# Autodesk Inventor assembly: Carrier Wirebonding Plate Assembly
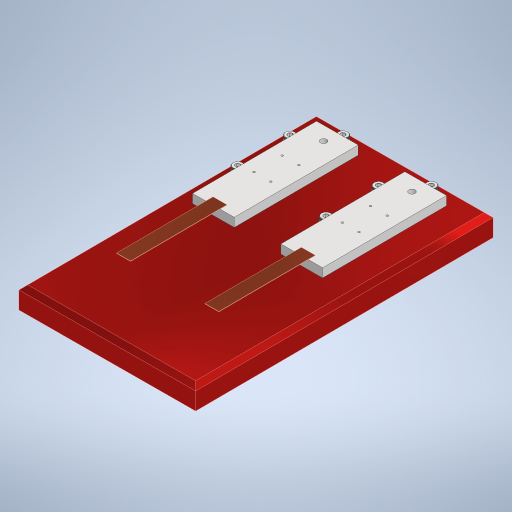
[picture p0: Inventor's stored thumbnail of the model, 512x512]
Saved by Autodesk Inventor 2023 (Build 270158000, 158)
## iProperties
Created: 2023-03-15
Part Number: Carrier Wirebonding Plate Assembly
Document SubType Name: Assembly
Designer: Caleb
Author: Caleb
## Documents named in this file (4)
- C:\Users\Caleb\Desktop\nebraska-silicon-lab\Hardware\TFPX\Carrier Wirebonding Plate\Carrier Wirebonding Plate Assembly.iam
- C:\Users\Caleb\Desktop\nebraska-silicon-lab\Hardware\TFPX\Carrier Wirebonding Plate\Carrier Wirebonding Plate.ipt
- C:\Users\Caleb\Desktop\nebraska-silicon-lab\Hardware\TFPX\Carrier Wirebonding Plate\Carrier Assembly.iam
- C:\Users\Caleb\Desktop\nebraska-silicon-lab\Hardware\TFPX\Carrier Wirebonding Plate\90128A212_Zinc-Plated Alloy Steel Socket Head Screw.ipt
## Components (9 placed, 3 different names)
1. Carrier Wirebonding Plate:1 — Mate:1, Angle:1, Insert:1, Insert:2, Insert:3, Insert:4, Insert:5, Insert:6, Mate:2, Angle:2
2. Carrier Assembly:1 [sub-assembly] — Mate:1, Angle:1, Tangent:1, Tangent:2, Tangent:3
3. 90128A212_Zinc-Plated Alloy Steel Socket Head Screw:1 — Insert:1, Tangent:2
4. 90128A212_Zinc-Plated Alloy Steel Socket Head Screw:2 — Insert:2, Tangent:1
5. 90128A212_Zinc-Plated Alloy Steel Socket Head Screw:3 — Insert:3, Tangent:3
6. 90128A212_Zinc-Plated Alloy Steel Socket Head Screw:4 — Insert:6, Tangent:4
7. 90128A212_Zinc-Plated Alloy Steel Socket Head Screw:5 — Insert:5, Tangent:5
8. 90128A212_Zinc-Plated Alloy Steel Socket Head Screw:6 — Insert:4
9. Carrier Assembly:2 [sub-assembly] — Mate:2, Angle:2, Tangent:4, Tangent:5
## Relationships (15: Insert 6, Tangent 5, Mate 2, Angle 2)
- Mate:1: Carrier Wirebonding Plate:1 ↔ Carrier Assembly:1
- Angle:1 (0 deg): Carrier Wirebonding Plate:1 ↔ Carrier Assembly:1
- Insert:1: Carrier Wirebonding Plate:1 ↔ 90128A212_Zinc-Plated Alloy Steel Socket Head Screw:1
- Insert:2: Carrier Wirebonding Plate:1 ↔ 90128A212_Zinc-Plated Alloy Steel Socket Head Screw:2
- Insert:3: Carrier Wirebonding Plate:1 ↔ 90128A212_Zinc-Plated Alloy Steel Socket Head Screw:3
- Tangent:1: Carrier Assembly:1 ↔ 90128A212_Zinc-Plated Alloy Steel Socket Head Screw:2
- Tangent:2: Carrier Assembly:1 ↔ 90128A212_Zinc-Plated Alloy Steel Socket Head Screw:1
- Tangent:3: Carrier Assembly:1 ↔ 90128A212_Zinc-Plated Alloy Steel Socket Head Screw:3
- Insert:4: Carrier Wirebonding Plate:1 ↔ 90128A212_Zinc-Plated Alloy Steel Socket Head Screw:6
- Insert:5: Carrier Wirebonding Plate:1 ↔ 90128A212_Zinc-Plated Alloy Steel Socket Head Screw:5
- Insert:6: Carrier Wirebonding Plate:1 ↔ 90128A212_Zinc-Plated Alloy Steel Socket Head Screw:4
- Mate:2: Carrier Wirebonding Plate:1 ↔ Carrier Assembly:2
- Angle:2 (0 deg): Carrier Wirebonding Plate:1 ↔ Carrier Assembly:2
- Tangent:4: 90128A212_Zinc-Plated Alloy Steel Socket Head Screw:4 ↔ Carrier Assembly:2
- Tangent:5: 90128A212_Zinc-Plated Alloy Steel Socket Head Screw:5 ↔ Carrier Assembly:2
